# Autodesk Inventor assembly: TW2A-001_CAM1
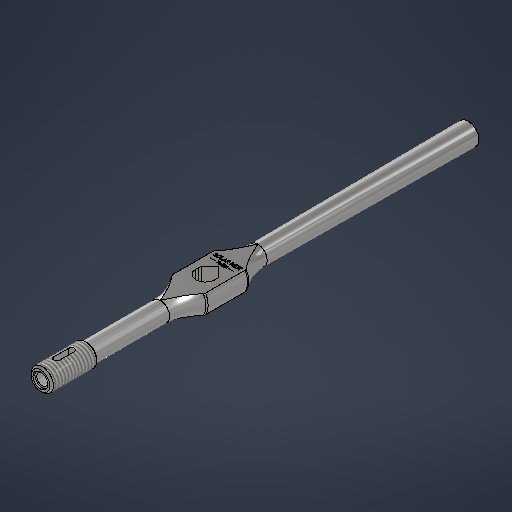
[picture p0: Inventor's stored thumbnail of the model, 512x512]
Saved by Autodesk Inventor 2025.3 (Build 293356000, 356)
## iProperties
Created: 2025-11-01
Part Number: TW2A-001_CAM1
Document SubType Name: Assembly
Designer: fablabadmin
Author: fablabadmin
## Documents named in this file (7)
- C:\Users\fablabadmin\Documents\_Benjamin_S\_3dCAD\_WEDU\TapWrench2A\TW2A-001_CAM1\TW2A-001_CAM1.iam
- C:\Users\fablabadmin\Documents\_Benjamin_S\_3dCAD\_WEDU\TapWrench2A\TW2A-001.ipt
- C:\Users\fablabadmin\Documents\_Benjamin_S\_3dCAD\_WEDU\TapWrench2A\TW2A-001_CAM1\RoundStock.ipt
- C:\Users\fablabadmin\Documents\_Benjamin_S\_3dCAD\_Config\KemmlerVise\OP1-KemmlerVise.iam
- C:\Users\fablabadmin\Documents\Inventor\Content Center Files\R2024\en-US\en-US\StandardJaw\JawSTD-Aluminum 6061.ipt
- C:\Users\fablabadmin\Documents\Inventor\Content Center Files\R2024\en-US\en-US\V-Block\vBlock.ipt
- C:\Users\fablabadmin\Documents\_Benjamin_S\_3dCAD\_Config\KemmlerVise\OP2-KemmlerVise.iam
## Components (10 placed, 6 different names)
1. TW2A-001:1 — Mate:5, Flush:2, Mate:6, Flush:6, Flush:10
2. RoundStock:1 — Mate:5, Flush:2, Flush:3, Tangent:1, Tangent:2, Tangent:3, Tangent:4, Tangent:5, Tangent:6
3. V-Block-Steel vBlock:1 — Tangent:1, Tangent:2, Angle:1, Mate:11, Mate:12, Flush:7
4. JawStandard JawSTD-Aluminum 6061:2 — Mate:9, Flush:5, Tangent:3
5. JawStandard JawSTD-Aluminum 6061:1 — Mate:8, Flush:4, Flush:5, Mate:10, Flush:6, Mate:12, Flush:7
6. OP1-KemmlerVise:1 [sub-assembly] — Mate:8, Mate:9, Flush:4, Mate:10, Mate:11
7. OP2-KemmlerVise:1 [sub-assembly] — Mate:13, Mate:14, Flush:8, Mate:15, Mate:17
8. JawStandard JawSTD-Aluminum 6061:3 — Mate:13, Flush:8, Flush:9, Mate:15, Mate:16, Flush:10, Flush:11
9. JawStandard JawSTD-Aluminum 6061:4 — Mate:14, Flush:9, Tangent:6
10. V-Block-Steel vBlock:2 — Tangent:4, Tangent:5, Angle:2, Mate:16, Mate:17, Flush:11
## Relationships (31: Mate 13, Flush 10, Tangent 6, Angle 2)
- Mate:5: TW2A-001:1 ↔ RoundStock:1
- Flush:2: TW2A-001:1 ↔ RoundStock:1
- Flush:3: RoundStock:1
- Mate:6: TW2A-001:1
- Mate:7
- Mate:8: JawStandard JawSTD-Aluminum 6061:1 ↔ OP1-KemmlerVise:1
- Mate:9: JawStandard JawSTD-Aluminum 6061:2 ↔ OP1-KemmlerVise:1
- Flush:4: JawStandard JawSTD-Aluminum 6061:1 ↔ OP1-KemmlerVise:1
- Flush:5: JawStandard JawSTD-Aluminum 6061:2 ↔ JawStandard JawSTD-Aluminum 6061:1
- Mate:10: JawStandard JawSTD-Aluminum 6061:1 ↔ OP1-KemmlerVise:1
- Tangent:1: RoundStock:1 ↔ V-Block-Steel vBlock:1
- Tangent:2: RoundStock:1 ↔ V-Block-Steel vBlock:1
- Angle:1 (0 deg): V-Block-Steel vBlock:1
- Mate:11 (13 mm): V-Block-Steel vBlock:1 ↔ OP1-KemmlerVise:1
- Flush:6 (135 mm): TW2A-001:1 ↔ JawStandard JawSTD-Aluminum 6061:1
- Mate:12: V-Block-Steel vBlock:1 ↔ JawStandard JawSTD-Aluminum 6061:1
- Tangent:3: RoundStock:1 ↔ JawStandard JawSTD-Aluminum 6061:2
- Flush:7: V-Block-Steel vBlock:1 ↔ JawStandard JawSTD-Aluminum 6061:1
- Mate:13: OP2-KemmlerVise:1 ↔ JawStandard JawSTD-Aluminum 6061:3
- Mate:14: OP2-KemmlerVise:1 ↔ JawStandard JawSTD-Aluminum 6061:4
- Flush:8: OP2-KemmlerVise:1 ↔ JawStandard JawSTD-Aluminum 6061:3
- Flush:9: JawStandard JawSTD-Aluminum 6061:3 ↔ JawStandard JawSTD-Aluminum 6061:4
- Mate:15: OP2-KemmlerVise:1 ↔ JawStandard JawSTD-Aluminum 6061:3
- Tangent:4: RoundStock:1 ↔ V-Block-Steel vBlock:2
- Tangent:5: RoundStock:1 ↔ V-Block-Steel vBlock:2
- Angle:2 (0 deg): V-Block-Steel vBlock:2
- Mate:16: JawStandard JawSTD-Aluminum 6061:3 ↔ V-Block-Steel vBlock:2
- Tangent:6: RoundStock:1 ↔ JawStandard JawSTD-Aluminum 6061:4
- Mate:17 (13 mm): OP2-KemmlerVise:1 ↔ V-Block-Steel vBlock:2
- Flush:10 (135 mm): TW2A-001:1 ↔ JawStandard JawSTD-Aluminum 6061:3
- Flush:11: JawStandard JawSTD-Aluminum 6061:3 ↔ V-Block-Steel vBlock:2
